# Autodesk Inventor assembly: клешня сбока
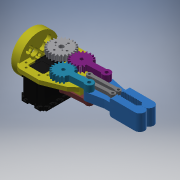
[picture p0: Inventor's stored thumbnail of the model, 180x180]
Saved by Autodesk Inventor 2019 (Build 230136000, 136)
## iProperties
Created: 2019-08-18
Part Number: клешня сбока
Material: Типовые
Document SubType Name: Assembly
Designer: Петров Иван
Mass: 103.83 g
Surface Area: 471.759 cm^2
Volume: 98.2815 cm^3
Density: 1.05645 g/cm^3
Author: Петров Иван
## Documents named in this file (10)
- E:\IVAN\Ivan_desktop\Kvantorium\Projects\optimal_gripper\hardware\КВ33.044.200 - Сборка зажима.iam
- E:\IVAN\Ivan_desktop\Kvantorium\Projects\optimal_gripper\hardware\КВ33.044.201 - Опора зажимного механизма.ipt
- E:\IVAN\Ivan_desktop\Kvantorium\Projects\optimal_gripper\hardware\Стандартные изделия\Сервомотор Dynamixel AX-12A\AX-12.iam
- E:\IVAN\Ivan_desktop\Kvantorium\Projects\optimal_gripper\hardware\Стандартные изделия\Подшипник 4x8x3.ipt
- E:\IVAN\Ivan_desktop\Kvantorium\Projects\optimal_gripper\hardware\КВ33.044.102 - Колесо зубчатое сервомотора.ipt
- E:\IVAN\Ivan_desktop\Kvantorium\Projects\optimal_gripper\hardware\КВ33.044.205 - Рычаг приводной 17 зубьев.ipt
- E:\IVAN\Ivan_desktop\Kvantorium\Projects\optimal_gripper\hardware\КВ33.044.206 - Рычаг приводной 16 зубьев.ipt
- E:\IVAN\Ivan_desktop\Kvantorium\Projects\optimal_gripper\hardware\КВ33.044.202 -Прихват.ipt
- E:\IVAN\Ivan_desktop\Kvantorium\Projects\optimal_gripper\hardware\КВ33.044.203 - Рычаг толстый.ipt
- E:\IVAN\Ivan_desktop\Kvantorium\Projects\optimal_gripper\hardware\КВ33.044.204 -Рычаг тонкий.ipt
## Components (23 placed, 9 different names)
1. КВ33.044.201 - Опора зажимного механизма:1 — Совмещение:40, Совмещение:42, Совмещение:50, Совмещение:51, Совмещение:52, Совмещение:53, Совмещение:54, Совмещение:55, Совмещение:56, Совмещение:57, Совмещение:58, Совмещение:61, Совмещение:62, Совмещение:63, Совмещение:64, Совмещение:65, Совмещение:66, Совмещение:67, Совмещение:68, Совмещение:73, Совмещение:75, Совмещение:81, Совмещение:84, Совмещение:87, Совмещение:90, Совмещение:93, Совмещение:96
2. AX-12:1 [sub-assembly] — Совмещение:40, Совмещение:42, Совмещение:50, Совмещение:59, Совмещение:60
3. Подшипник 4x8x3:1 — Совмещение:53, Совмещение:54, Совмещение:85
4. Подшипник 4x8x3:2 — Совмещение:55, Совмещение:56, Совмещение:91
5. Подшипник 4x8x3:3 — Совмещение:51, Совмещение:52, Совмещение:82
6. Подшипник 4x8x3:4 — Совмещение:57, Совмещение:58, Совмещение:88
7. КВ33.044.102 - Колесо зубчатое сервомотора:1 — Совмещение:59, Совмещение:60
8. КВ33.044.205 - Рычаг приводной 17 зубьев:1 — Совмещение:69, Совмещение:70, Совмещение:76, Совмещение:77, Совмещение:78
9. КВ33.044.206 - Рычаг приводной 16 зубьев:1 — Совмещение:71, Совмещение:72, Совмещение:74, Совмещение:79, Совмещение:80
10. Подшипник 4x8x3:5 — Совмещение:61, Совмещение:62, Совмещение:74
11. Подшипник 4x8x3:6 — Совмещение:63, Совмещение:64, Совмещение:76
12. Подшипник 4x8x3:8 — Совмещение:65, Совмещение:66, Совмещение:97
13. Подшипник 4x8x3:9 — Совмещение:67, Совмещение:68, Совмещение:94
14. Подшипник 4x8x3:10 — Совмещение:69, Совмещение:70, Совмещение:75
15. Подшипник 4x8x3:11 — Совмещение:71, Совмещение:72, Совмещение:73
16. КВ33.044.202 -Прихват:1 — Совмещение:77, Совмещение:78, Совмещение:86, Совмещение:92, Совмещение:98
17. КВ33.044.202 -Прихват:2 — Совмещение:79, Совмещение:80, Совмещение:83, Совмещение:89, Совмещение:95
18. КВ33.044.203 - Рычаг толстый:1 — Совмещение:81, Совмещение:82, Совмещение:83
19. КВ33.044.203 - Рычаг толстый:2 — Совмещение:84, Совмещение:85, Совмещение:86
20. КВ33.044.204 -Рычаг тонкий:1 — Совмещение:96, Совмещение:97, Совмещение:98
21. КВ33.044.204 -Рычаг тонкий:2 — Совмещение:90, Совмещение:91, Совмещение:92
22. КВ33.044.204 -Рычаг тонкий:3 — Совмещение:87, Совмещение:88, Совмещение:89
23. КВ33.044.204 -Рычаг тонкий:4 — Совмещение:93, Совмещение:94, Совмещение:95
## Relationships (51: Mate 51)
- Совмещение:40 [Mate]: КВ33.044.201 - Опора зажимного механизма:1 ↔ AX-12:1
- Совмещение:42 [Mate]: КВ33.044.201 - Опора зажимного механизма:1 ↔ AX-12:1
- Совмещение:50 [Mate]: КВ33.044.201 - Опора зажимного механизма:1 ↔ AX-12:1
- Совмещение:51 [Mate]: КВ33.044.201 - Опора зажимного механизма:1 ↔ Подшипник 4x8x3:3
- Совмещение:52 [Mate]: КВ33.044.201 - Опора зажимного механизма:1 ↔ Подшипник 4x8x3:3
- Совмещение:53 [Mate]: КВ33.044.201 - Опора зажимного механизма:1 ↔ Подшипник 4x8x3:1
- Совмещение:54 [Mate]: КВ33.044.201 - Опора зажимного механизма:1 ↔ Подшипник 4x8x3:1
- Совмещение:55 [Mate]: КВ33.044.201 - Опора зажимного механизма:1 ↔ Подшипник 4x8x3:2
- Совмещение:56 [Mate]: КВ33.044.201 - Опора зажимного механизма:1 ↔ Подшипник 4x8x3:2
- Совмещение:57 [Mate]: КВ33.044.201 - Опора зажимного механизма:1 ↔ Подшипник 4x8x3:4
- Совмещение:58 [Mate]: КВ33.044.201 - Опора зажимного механизма:1 ↔ Подшипник 4x8x3:4
- Совмещение:59 [Mate]: AX-12:1 ↔ КВ33.044.102 - Колесо зубчатое сервомотора:1
- Совмещение:60 [Mate]: AX-12:1 ↔ КВ33.044.102 - Колесо зубчатое сервомотора:1
- Совмещение:61 [Mate]: КВ33.044.201 - Опора зажимного механизма:1 ↔ Подшипник 4x8x3:5
- Совмещение:62 [Mate]: КВ33.044.201 - Опора зажимного механизма:1 ↔ Подшипник 4x8x3:5
- Совмещение:63 [Mate]: КВ33.044.201 - Опора зажимного механизма:1 ↔ Подшипник 4x8x3:6
- Совмещение:64 [Mate]: КВ33.044.201 - Опора зажимного механизма:1 ↔ Подшипник 4x8x3:6
- Совмещение:65 [Mate]: КВ33.044.201 - Опора зажимного механизма:1 ↔ Подшипник 4x8x3:8
- Совмещение:66 [Mate]: КВ33.044.201 - Опора зажимного механизма:1 ↔ Подшипник 4x8x3:8
- Совмещение:67 [Mate]: КВ33.044.201 - Опора зажимного механизма:1 ↔ Подшипник 4x8x3:9
- Совмещение:68 [Mate]: КВ33.044.201 - Опора зажимного механизма:1 ↔ Подшипник 4x8x3:9
- Совмещение:69 [Mate]: КВ33.044.205 - Рычаг приводной 17 зубьев:1 ↔ Подшипник 4x8x3:10
- Совмещение:70 [Mate]: КВ33.044.205 - Рычаг приводной 17 зубьев:1 ↔ Подшипник 4x8x3:10
- Совмещение:71 [Mate]: КВ33.044.206 - Рычаг приводной 16 зубьев:1 ↔ Подшипник 4x8x3:11
- Совмещение:72 [Mate]: КВ33.044.206 - Рычаг приводной 16 зубьев:1 ↔ Подшипник 4x8x3:11
- Совмещение:73 [Mate]: КВ33.044.201 - Опора зажимного механизма:1 ↔ Подшипник 4x8x3:11
- Совмещение:74 [Mate]: КВ33.044.206 - Рычаг приводной 16 зубьев:1 ↔ Подшипник 4x8x3:5
- Совмещение:75 [Mate]: КВ33.044.201 - Опора зажимного механизма:1 ↔ Подшипник 4x8x3:10
- Совмещение:76 [Mate]: КВ33.044.205 - Рычаг приводной 17 зубьев:1 ↔ Подшипник 4x8x3:6
- Совмещение:77 [Mate]: КВ33.044.205 - Рычаг приводной 17 зубьев:1 ↔ КВ33.044.202 -Прихват:1
- Совмещение:78 [Mate]: КВ33.044.205 - Рычаг приводной 17 зубьев:1 ↔ КВ33.044.202 -Прихват:1
- Совмещение:79 [Mate]: КВ33.044.206 - Рычаг приводной 16 зубьев:1 ↔ КВ33.044.202 -Прихват:2
- Совмещение:80 [Mate]: КВ33.044.206 - Рычаг приводной 16 зубьев:1 ↔ КВ33.044.202 -Прихват:2
- Совмещение:81 [Mate]: КВ33.044.201 - Опора зажимного механизма:1 ↔ КВ33.044.203 - Рычаг толстый:1
- Совмещение:82 [Mate]: Подшипник 4x8x3:3 ↔ КВ33.044.203 - Рычаг толстый:1
- Совмещение:83 [Mate]: КВ33.044.202 -Прихват:2 ↔ КВ33.044.203 - Рычаг толстый:1
- Совмещение:84 [Mate]: КВ33.044.201 - Опора зажимного механизма:1 ↔ КВ33.044.203 - Рычаг толстый:2
- Совмещение:85 [Mate]: Подшипник 4x8x3:1 ↔ КВ33.044.203 - Рычаг толстый:2
- Совмещение:86 [Mate]: КВ33.044.202 -Прихват:1 ↔ КВ33.044.203 - Рычаг толстый:2
- Совмещение:87 [Mate]: КВ33.044.201 - Опора зажимного механизма:1 ↔ КВ33.044.204 -Рычаг тонкий:3
- Совмещение:88 [Mate]: Подшипник 4x8x3:4 ↔ КВ33.044.204 -Рычаг тонкий:3
- Совмещение:89 [Mate]: КВ33.044.202 -Прихват:2 ↔ КВ33.044.204 -Рычаг тонкий:3
- Совмещение:90 [Mate]: КВ33.044.201 - Опора зажимного механизма:1 ↔ КВ33.044.204 -Рычаг тонкий:2
- Совмещение:91 [Mate]: Подшипник 4x8x3:2 ↔ КВ33.044.204 -Рычаг тонкий:2
- Совмещение:92 [Mate]: КВ33.044.202 -Прихват:1 ↔ КВ33.044.204 -Рычаг тонкий:2
- Совмещение:93 [Mate]: КВ33.044.201 - Опора зажимного механизма:1 ↔ КВ33.044.204 -Рычаг тонкий:4
- Совмещение:94 [Mate]: Подшипник 4x8x3:9 ↔ КВ33.044.204 -Рычаг тонкий:4
- Совмещение:95 [Mate]: КВ33.044.202 -Прихват:2 ↔ КВ33.044.204 -Рычаг тонкий:4
- Совмещение:96 [Mate]: КВ33.044.201 - Опора зажимного механизма:1 ↔ КВ33.044.204 -Рычаг тонкий:1
- Совмещение:97 [Mate]: Подшипник 4x8x3:8 ↔ КВ33.044.204 -Рычаг тонкий:1
- Совмещение:98 [Mate]: КВ33.044.202 -Прихват:1 ↔ КВ33.044.204 -Рычаг тонкий:1
